# Autodesk Inventor assembly: Flywheel
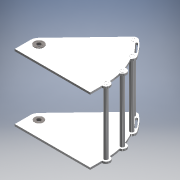
[picture p0: Inventor's stored thumbnail of the model, 180x180]
Saved by Autodesk Inventor 2018 (Build 220112000, 112)
## iProperties
Created: 2020-01-19
Part Number: Flywheel
Document SubType Name: Assembly
Designer: Victor
Author: Victor
## Documents named in this file (4)
- E:\Downloads\GrabCAD\Infinite Recharge 2020\Build season\Flywheel\Flywheel.iam
- E:\Downloads\GrabCAD\Infinite Recharge 2020\Build season\Flywheel\Hood panel.ipt
- E:\Downloads\GrabCAD\Infinite Recharge 2020\Build season\Flywheel\Hood rod.ipt
- E:\Downloads\GrabCAD\Deep Space 2019\Build Season\Chassis\217-2731_0_500_flanged_bearing.ipt
## Components (8 placed, 3 different names)
1. Hood panel:1 — Insert:1, Insert:2, Insert:3, Insert:4, Insert:10
2. Hood panel:2 — Insert:5, Insert:6, Insert:7, Insert:8, Insert:9
3. Hood rod:1 — Insert:2, Insert:6
4. Hood rod:2 — Insert:3, Insert:7
5. Hood rod:3 — Insert:4, Insert:8
6. Hood rod:4 — Insert:1, Insert:5
7. 217-2731_0_500_flanged_bearing:1 — Insert:9
8. 217-2731_0_500_flanged_bearing:2 — Insert:10
## Relationships (10: Insert 10)
- Insert:1: Hood panel:1 ↔ Hood rod:4
- Insert:2: Hood panel:1 ↔ Hood rod:1
- Insert:3: Hood panel:1 ↔ Hood rod:2
- Insert:4: Hood panel:1 ↔ Hood rod:3
- Insert:5: Hood panel:2 ↔ Hood rod:4
- Insert:6: Hood panel:2 ↔ Hood rod:1
- Insert:7: Hood panel:2 ↔ Hood rod:2
- Insert:8: Hood panel:2 ↔ Hood rod:3
- Insert:9: Hood panel:2 ↔ 217-2731_0_500_flanged_bearing:1
- Insert:10: Hood panel:1 ↔ 217-2731_0_500_flanged_bearing:2
